# Autodesk Inventor assembly: base_assembly
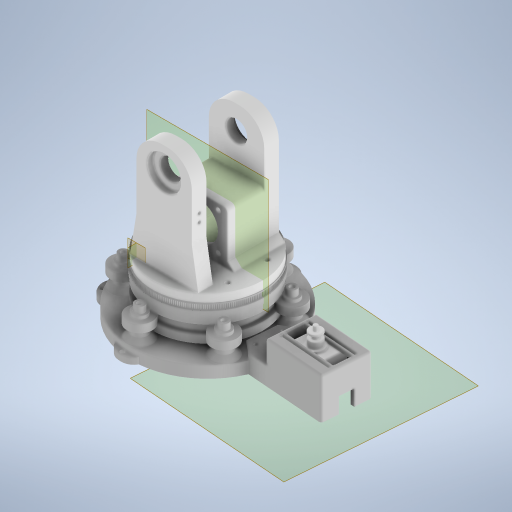
[picture p0: Inventor's stored thumbnail of the model, 512x512]
Saved by Autodesk Inventor 2024 (Build 280153000, 153)
## iProperties
Created: 2024-02-08
Part Number: base_assembly
Document SubType Name: Assembly
Designer: MaartenGeorgesBuelen
Author: MaartenGeorgesBuelen
## Documents named in this file (12)
- C:\Users\MaartenGeorgesBuelen\Documents\Inventor\robot arm\base-new\base_assembly.iam
- C:\Users\MaartenGeorgesBuelen\Documents\Inventor\robot arm\base-new\base.ipt
- C:\Users\MaartenGeorgesBuelen\Documents\Inventor\robot arm\base-new\base-top-plate.ipt
- C:\Users\MaartenGeorgesBuelen\Documents\Inventor\robot arm\hardware\base_bolt.ipt
- C:\Users\MaartenGeorgesBuelen\Documents\Inventor\robot arm\hardware\base_bolt_bearing.ipt
- C:\Users\MaartenGeorgesBuelen\Documents\Inventor\robot arm\hardware\base_bearing_Circle.ipt
- C:\Users\MaartenGeorgesBuelen\Documents\Inventor\robot arm\base-new\base-bottom-plate.ipt
- C:\Users\MaartenGeorgesBuelen\Documents\Inventor\robot arm\hardware\base-bearing-cap.ipt
- C:\Users\MaartenGeorgesBuelen\Documents\Inventor\robot arm\hardware\pulley-140mm.ipt
- C:\Users\MaartenGeorgesBuelen\Documents\Inventor\robot arm\base-new\base-stepper-holder.ipt
- C:\Users\MaartenGeorgesBuelen\Documents\Inventor\robot arm\motors\stepper motor.ipt
- C:\Users\MaartenGeorgesBuelen\Documents\Inventor\robot arm\hardware\pulley-small.ipt
## Components (27 placed, 11 different names)
1. base:1 — Mate:41, Mate:42, Mate:43
2. base-top-plate:1 — Mate:3, Flush:3, Mate:4, Tangent:1, Mate:7, Mate:8, Mate:9, Mate:10, Mate:11, Tangent:2, Tangent:3, Tangent:4, Tangent:5, Tangent:6, Tangent:7, Mate:36, Mate:37, Mate:39, Mate:41, Mate:42
3. base-bottom-plate:1 — Mate:12, Mate:13, Mate:14, Mate:15, Mate:16, Mate:17, Flush:7, Flush:8, Mate:45, Mate:46
4. pulley-140mm:1 — Mate:37, Mate:38, Mate:39, Mate:43
5. base-stepper-holder:1 — Flush:7, Mate:45, Mate:46
6. stepper motor:1 — Mate:44, Flush:8
7. pulley-small:1 — Mate:44
8. base-bearing-cap:2 — Mate:20, Mate:32, Mate:33
9. base-bearing-cap:3 — Mate:24, Mate:30, Mate:31
10. base-bearing-cap:4 — Mate:22, Mate:34, Mate:35
11. base-bearing-cap:5 — Mate:21, Mate:26, Mate:27
12. base-bearing-cap:6 — Mate:23, Mate:28, Mate:29
13. base_bolt:3 — Mate:26, Mate:27
14. base_bolt:4 — Mate:28, Mate:29
15. base_bolt:5 — Mate:30, Mate:31
16. base_bolt:6 — Mate:32, Mate:33
17. base_bolt:7 — Mate:34, Mate:35
18. base_bolt:1 — Mate:3, Flush:3, Mate:5, Mate:38
19. base_bolt:2 — Mate:19, Mate:25
20. base-bearing-cap:1 — Flush:6, Mate:19, Mate:25
21. base_bearing_Circle:1 — Tangent:1, Tangent:7, Mate:17, Mate:24, Mate:36
22. base_bearing_Circle:2 — Mate:7, Tangent:6, Mate:15, Mate:23
23. base_bearing_Circle:3 — Mate:9, Tangent:4, Mate:12, Flush:6
24. base_bearing_Circle:4 — Mate:8, Tangent:5, Mate:14, Mate:21
25. base_bearing_Circle:5 — Mate:10, Tangent:3, Mate:13, Mate:20
26. base_bearing_Circle:6 — Mate:11, Tangent:2, Mate:16, Mate:22
27. base_bolt_bearing:1 — Mate:4, Mate:5
## Relationships (52: Mate 41, Tangent 7, Flush 4)
- Mate:3: base-top-plate:1 ↔ base_bolt:1
- Flush:3 (10 mm): base-top-plate:1 ↔ base_bolt:1
- Mate:4: base-top-plate:1 ↔ base_bolt_bearing:1
- Mate:5: base_bolt:1 ↔ base_bolt_bearing:1
- Tangent:1: base-top-plate:1 ↔ base_bearing_Circle:1
- Mate:7: base-top-plate:1 ↔ base_bearing_Circle:2
- Mate:8: base-top-plate:1 ↔ base_bearing_Circle:4
- Mate:9: base-top-plate:1 ↔ base_bearing_Circle:3
- Mate:10: base-top-plate:1 ↔ base_bearing_Circle:5
- Mate:11: base-top-plate:1 ↔ base_bearing_Circle:6
- Tangent:2: base-top-plate:1 ↔ base_bearing_Circle:6
- Tangent:3: base-top-plate:1 ↔ base_bearing_Circle:5
- Tangent:4: base-top-plate:1 ↔ base_bearing_Circle:3
- Tangent:5: base-top-plate:1 ↔ base_bearing_Circle:4
- Tangent:6: base-top-plate:1 ↔ base_bearing_Circle:2
- Tangent:7: base-top-plate:1 ↔ base_bearing_Circle:1
- Mate:12: base-bottom-plate:1 ↔ base_bearing_Circle:3
- Mate:13: base-bottom-plate:1 ↔ base_bearing_Circle:5
- Mate:14: base-bottom-plate:1 ↔ base_bearing_Circle:4
- Mate:15: base-bottom-plate:1 ↔ base_bearing_Circle:2
- Mate:16: base-bottom-plate:1 ↔ base_bearing_Circle:6
- Mate:17: base-bottom-plate:1 ↔ base_bearing_Circle:1
- Flush:6: base-bearing-cap:1 ↔ base_bearing_Circle:3
- Mate:19: base_bolt:2 ↔ base-bearing-cap:1
- Mate:20: base-bearing-cap:2 ↔ base_bearing_Circle:5
- Mate:21: base-bearing-cap:5 ↔ base_bearing_Circle:4
- Mate:22: base-bearing-cap:4 ↔ base_bearing_Circle:6
- Mate:23: base-bearing-cap:6 ↔ base_bearing_Circle:2
- Mate:24: base-bearing-cap:3 ↔ base_bearing_Circle:1
- Mate:25: base_bolt:2 ↔ base-bearing-cap:1
- Mate:26: base-bearing-cap:5 ↔ base_bolt:3
- Mate:27: base-bearing-cap:5 ↔ base_bolt:3
- Mate:28: base-bearing-cap:6 ↔ base_bolt:4
- Mate:29: base-bearing-cap:6 ↔ base_bolt:4
- Mate:30: base-bearing-cap:3 ↔ base_bolt:5
- Mate:31: base-bearing-cap:3 ↔ base_bolt:5
- Mate:32: base-bearing-cap:2 ↔ base_bolt:6
- Mate:33: base-bearing-cap:2 ↔ base_bolt:6
- Mate:34: base-bearing-cap:4 ↔ base_bolt:7
- Mate:35: base-bearing-cap:4 ↔ base_bolt:7
- Mate:36: base-top-plate:1 ↔ base_bearing_Circle:1
- Mate:37: base-top-plate:1 ↔ pulley-140mm:1
- Mate:38: pulley-140mm:1 ↔ base_bolt:1
- Mate:39: base-top-plate:1 ↔ pulley-140mm:1
- Mate:41: base:1 ↔ base-top-plate:1
- Mate:42: base:1 ↔ base-top-plate:1
- Mate:43: base:1 ↔ pulley-140mm:1
- Flush:7: base-bottom-plate:1 ↔ base-stepper-holder:1
- Mate:44: stepper motor:1 ↔ pulley-small:1
- Flush:8: base-bottom-plate:1 ↔ stepper motor:1
- Mate:45: base-bottom-plate:1 ↔ base-stepper-holder:1
- Mate:46: base-bottom-plate:1 ↔ base-stepper-holder:1
